# Autodesk Inventor assembly: slock
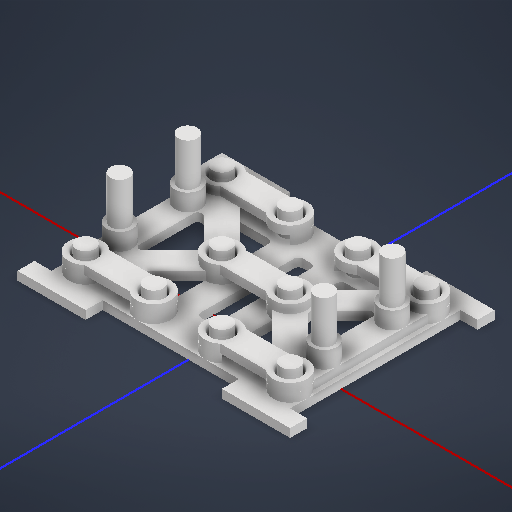
[picture p0: Inventor's stored thumbnail of the model, 512x512]
Saved by Autodesk Inventor 2025.4 (Build 294407000, 407)
## iProperties
Created: 2026-09-15
Part Number: slock
Document SubType Name: Assembly
Designer: User
Author: User
## Documents named in this file (4)
- G:\projects\primary\mechanical-computer\mechanics\lock\lock.iam
- G:\projects\primary\mechanical-computer\mechanics\links\link.ipt
- G:\projects\primary\mechanical-computer\mechanics\lock\bar.ipt
- G:\projects\primary\mechanical-computer\mechanics\lock\base.ipt
## Components (8 placed, 3 different names)
1. link:1 — Cylindrical:19, Mate:6, Cylindrical:21, Flush:2
2. bar:1 — Cylindrical:15, Cylindrical:16, Mate:2, Mate:4, Mate:5, Cylindrical:25
3. bar:2 — Cylindrical:18, Cylindrical:19, Mate:1, Mate:3, Mate:6, Mate:7, Cylindrical:24
4. link:2 — Mate:3, Cylindrical:24, Cylindrical:25
5. link:3 — Cylindrical:18, Mate:7, Cylindrical:20
6. link:4 — Cylindrical:15, Mate:4, Cylindrical:22
7. link:5 — Cylindrical:16, Mate:5, Cylindrical:23, Flush:1
8. base:1 — Mate:1, Mate:2, Cylindrical:20, Cylindrical:21, Cylindrical:22, Cylindrical:23, Flush:1, Flush:2
## Relationships (19: CylindricalJoint 10, Mate 7, Flush 2)
- Cylindrical:15: bar:1 ↔ link:4
- Cylindrical:16: bar:1 ↔ link:5
- Cylindrical:18: bar:2 ↔ link:3
- Cylindrical:19: link:1 ↔ bar:2
- Mate:1: bar:2 ↔ base:1
- Mate:2: bar:1 ↔ base:1
- Mate:3: bar:2 ↔ link:2
- Mate:4: bar:1 ↔ link:4
- Mate:5: bar:1 ↔ link:5
- Mate:6: link:1 ↔ bar:2
- Mate:7: bar:2 ↔ link:3
- Cylindrical:20: link:3 ↔ base:1
- Cylindrical:21: link:1 ↔ base:1
- Cylindrical:22: link:4 ↔ base:1
- Cylindrical:23: link:5 ↔ base:1
- Cylindrical:24: bar:2 ↔ link:2
- Cylindrical:25: bar:1 ↔ link:2
- Flush:1 (-0.5 mm): link:5 ↔ base:1
- Flush:2 (0.5 mm): link:1 ↔ base:1
